# Autodesk Inventor assembly: MIRleft脚四半
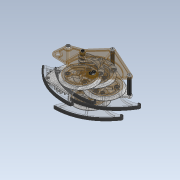
[picture p0: Inventor's stored thumbnail of the model, 180x180]
Saved by Autodesk Inventor 2020.2 (Build 242310000, 310)
## iProperties
Created: 2020-03-11
Part Number: MIRleft脚四半
Document SubType Name: Assembly
Designer: aoyama
Mass: 221.596 g
Surface Area: 1653.51 cm^2
Volume: 107.747 cm^3
Density: 2.05663 g/cm^3
Author: aoyam
## Documents named in this file (38)
- C:\Users\aoyam\Desktop\SRDC_local\Inventor\二年機\Geminiβ\脚\MIR達\MIRleft脚四半.iam
- C:\Users\aoyam\Desktop\SRDC_local\Inventor\二年機\Geminiβ\汎用部品\MIR達\MIRleftワッシャD8d6m0.5.ipt
- C:\Users\aoyam\Desktop\SRDC_local\Inventor\二年機\Geminiβ\汎用部品\MIR達\MIRleftワッシャD7d4m0.5.ipt
- C:\Users\aoyam\Desktop\SRDC_local\Inventor\二年機\Geminiβ\汎用部品\MIR達\MIRleftｍ2歯数17ギアd3.99.ipt
- C:\Users\aoyam\Desktop\SRDC_local\Inventor\二年機\Geminiβ\汎用部品\MIR達\MIRleftスペーサーM3L30アルミ.ipt
- C:\Users\aoyam\Desktop\SRDC_local\Inventor\二年機\Geminiβ\汎用部品\MIR達\MIRleftネジボタンM3L6.ipt
- C:\Users\aoyam\Desktop\SRDC_local\Inventor\二年機\Geminiβ\汎用部品\MIR達\MIRleftネジボタンM3L8.ipt
- C:\Users\aoyam\Desktop\SRDC_local\Inventor\二年機\Geminiβ\汎用部品\MIR達\MIRleftネジボタンM3L10.ipt
- C:\Users\aoyam\Desktop\SRDC_local\Inventor\二年機\Geminiβ\汎用部品\MIR達\MIRleftスペーサーM3L30樹脂.ipt
- C:\Users\aoyam\Desktop\SRDC_local\Inventor\二年機\Geminiβ\汎用部品\MIR達\MIRleftオイレスFd6D8L7.ipt
- C:\Users\aoyam\Desktop\SRDC_local\Inventor\二年機\Geminiβ\汎用部品\MIR達\MIRleftネジアルミM3L6.ipt
- C:\Users\aoyam\Desktop\SRDC_local\Inventor\二年機\Geminiβ\脚\MIR達\MIRleft脚フレーム外側後.ipt
- C:\Users\aoyam\Desktop\SRDC_local\Inventor\二年機\Geminiβ\脚\ネジクランク\MIR達\MIRleft脚一枚.iam
- C:\Users\aoyam\Desktop\SRDC_local\Inventor\二年機\Geminiβ\脚\ネジクランク\MIR達\MIRleftカムL4F.ipt
- C:\Users\aoyam\Desktop\SRDC_local\Inventor\二年機\Geminiβ\汎用部品\MIR達\MIRleftオイレスドライメットFd10D12L3.ipt
- C:\Users\aoyam\Desktop\SRDC_local\Inventor\二年機\Geminiβ\汎用部品\MIR達\MIRleftｍ2歯数25ギアネジ.ipt
- C:\Users\aoyam\Desktop\SRDC_local\Inventor\二年機\Geminiβ\脚\ネジクランク\MIR達\MIRleftカムL3.ipt
- C:\Users\aoyam\Desktop\SRDC_local\Inventor\二年機\Geminiβ\汎用部品\MIR達\MIRleftオイレスドライメットFd10D12L4.ipt
- C:\Users\aoyam\Desktop\SRDC_local\Inventor\二年機\Geminiβ\脚\ネジクランク\MIR達\MIRleftカムL4.ipt
- C:\Users\aoyam\Desktop\SRDC_local\Inventor\二年機\Geminiβ\汎用部品\MIR達\MIRleftネジキャップM3L45.ipt
- C:\Users\aoyam\Desktop\SRDC_local\Inventor\二年機\Geminiβ\汎用部品\MIR達\MIRleftナットナイロンM3.ipt
- C:\Users\aoyam\Desktop\SRDC_local\Inventor\二年機\Geminiβ\汎用部品\MIR達\MIRleftスペーサーM3L40アルミ.ipt
- C:\Users\aoyam\Desktop\SRDC_local\Inventor\二年機\Geminiβ\汎用部品\MIR達\MIRleftネジ超極低頭M3L4.ipt
- C:\Users\aoyam\Desktop\SRDC_local\Inventor\二年機\Geminiβ\汎用部品\MIR達\MIRleftネジキャップM3L15.ipt
- C:\Users\aoyam\Desktop\SRDC_local\Inventor\二年機\Geminiβ\脚\MIR達\MIRleft脚フレーム内側後改.ipt
- C:\Users\aoyam\Desktop\SRDC_local\Inventor\二年機\Geminiβ\汎用部品\ベアリングFd4D11B4.ipt
- C:\Users\aoyam\Desktop\SRDC_local\Inventor\二年機\Geminiβ\汎用部品\オイレスFd6D8L4.ipt
- C:\Users\aoyam\Desktop\SRDC_local\Inventor\二年機\Geminiβ\汎用部品\ベアリングFd6D12B4.ipt
- C:\Users\aoyam\Desktop\SRDC_local\Inventor\二年機\Geminiβ\汎用部品\ワッシャD8d6m0.5.ipt
- C:\Users\aoyam\Desktop\SRDC_local\Inventor\二年機\Geminiβ\汎用部品\ｍ2歯数14ギアd12.ipt
- C:\Users\aoyam\Desktop\SRDC_local\Inventor\二年機\Geminiβ\汎用部品\ワッシャD10d6m0.3.ipt
- C:\Users\aoyam\Desktop\SRDC_local\Inventor\二年機\Geminiβ\汎用部品\オイレス外径8内径6L3.ipt
- C:\Users\aoyam\Desktop\SRDC_local\Inventor\二年機\Geminiβ\脚\MIRright脚ギアトレイン2.ipt
- C:\Users\aoyam\Desktop\SRDC_local\Inventor\二年機\Geminiβ\汎用部品\スペーサー中空M3L5樹脂.ipt
- C:\Users\aoyam\Desktop\SRDC_local\Inventor\二年機\Geminiβ\汎用部品\スペーサー中空M3L4樹脂.ipt
- C:\Users\aoyam\Desktop\SRDC_local\Inventor\二年機\Geminiβ\汎用部品\ネジ皿M3L8.ipt
- C:\Users\aoyam\Desktop\SRDC_local\Inventor\二年機\Geminiβ\汎用部品\ポリスラd6D14t0.25.ipt
- C:\Users\aoyam\Desktop\SRDC_local\Inventor\二年機\Geminiβ\汎用部品\平行ピンD4L12.ipt
## Components (61 placed, 37 different names)
1. MIRleftワッシャD7d4m0.5:1 — 挿入:9, 挿入:82
2. MIRleftｍ2歯数17ギアd3.99:1 — 挿入:9, 挿入:11
3. MIRleftワッシャD7d4m0.5:2 — 挿入:11, 挿入:81
4. MIRleftスペーサーM3L30アルミ:1 — 挿入:93, メイト:9, メイト:10, メイト:11, メイト:12, メイト:9, 挿入:73
5. MIRleftネジボタンM3L6:1 — 挿入:74
6. MIRleftネジボタンM3L8:1 — 挿入:97, メイト:9
7. MIRleftネジボタンM3L10:1 — 挿入:99
8. MIRleftネジボタンM3L10:2 — 挿入:97
9. MIRleftネジボタンM3L10:3 — 挿入:98
10. MIRleftスペーサーM3L30樹脂:1 — 挿入:71
11. MIRleftスペーサーM3L30樹脂:2 — 挿入:72, 挿入:77
12. MIRleftオイレスFd6D8L7:1 — 挿入:136, 挿入:137
13. MIRleftオイレスFd6D8L7:2 — 挿入:134
14. MIRleftオイレスFd6D8L7:3 — 挿入:135
15. MIRleftオイレスFd6D8L7:4 — 挿入:133
16. MIRleftワッシャD8d6m0.5:3 — 挿入:93, 挿入:129
17. MIRleftワッシャD8d6m0.5:4 — 挿入:130
18. MIRleftワッシャD8d6m0.5:5 — 挿入:129
19. MIRleftネジアルミM3L6:1 — 挿入:75
20. MIRleftネジアルミM3L6:2 — 挿入:76
21. MIRleftネジアルミM3L6:3 — 挿入:98
22. MIRleftネジアルミM3L6:4 — 挿入:99
23. MIRleft脚フレーム外側後:1 — 挿入:99, 挿入:98, 挿入:97, メイト:1, 挿入:111, 挿入:124, 挿入:77
24. MIRleft脚一枚:1 [sub-assembly] — 挿入:136, メイト:9, メイト:1, 挿入:104, 挿入:103, 挿入:110, 挿入:109
25. MIRleft脚一枚:2 [sub-assembly] — 挿入:135, メイト:10, 挿入:104, 挿入:103, 挿入:106, 挿入:105
26. MIRleft脚一枚:3 [sub-assembly] — 挿入:134, メイト:11, 挿入:106, 挿入:105, 挿入:108, 挿入:107
27. MIRleft脚一枚:4 [sub-assembly] — 挿入:133, メイト:12, 挿入:108, 挿入:107, メイト:6, メイト:7
28. MIRleftカムL4F:1 — 挿入:111, 挿入:110, 挿入:109, 挿入:112, 挿入:119, 挿入:120
29. MIRleftオイレスドライメットFd10D12L3:1 — 挿入:112
30. MIRleftｍ2歯数25ギアネジ:1 — メイト:6, 挿入:114, 挿入:116, 挿入:115, 挿入:78
31. MIRleftオイレスドライメットFd10D12L3:2 — 挿入:114
32. MIRleftカムL3:1 — 挿入:116, 挿入:115, 挿入:121, 挿入:122
33. MIRleftオイレスドライメットFd10D12L4:1 — 挿入:118, 挿入:78, 挿入:79
34. MIRleftカムL4:1 — メイト:7, 挿入:118
35. MIRleftネジキャップM3L45:1 — 挿入:119, メイト:10
36. MIRleftネジキャップM3L45:2 — 挿入:120
37. MIRleftナットナイロンM3:1 — 挿入:121, メイト:8, メイト:10
38. MIRleftナットナイロンM3:2 — メイト:8, 挿入:122
39. MIRleftスペーサーM3L40アルミ:1 — 挿入:124, 挿入:127, 挿入:100
40. MIRleftネジ超極低頭M3L4:1 — 挿入:127
41. MIRleftワッシャD8d6m0.5:6 — 挿入:137, 挿入:130
42. MIRleftネジキャップM3L15:1 — 挿入:101
43. MIRleft脚フレーム内側後改:1 — 挿入:71, 挿入:72, 挿入:73, 挿入:74, 挿入:75, 挿入:76, 挿入:79, 挿入:80, 挿入:83, 挿入:90, 挿入:91, 挿入:92, 挿入:93, 挿入:102
44. ベアリングFd4D11B4:1 — 挿入:82, 挿入:105
45. ベアリングFd4D11B4:2 — 挿入:80, 挿入:81
46. オイレスFd6D8L4:1 — 挿入:83, 挿入:84
47. ベアリングFd6D12B4:1 — 挿入:85, 挿入:86, 挿入:87
48. ワッシャD8d6m0.5:1 — 挿入:84, 挿入:85
49. ｍ2歯数14ギアd12:1 — 挿入:86
50. ワッシャD10d6m0.3:1 — 挿入:87, 挿入:88
51. オイレス外径8内径6L3:1 — 挿入:88, 挿入:89, 挿入:104
52. MIRright脚ギアトレイン2:1 — 挿入:89, 挿入:94, 挿入:95, 挿入:96, 挿入:97, 挿入:98, 挿入:99, 挿入:101
53. スペーサー中空M3L5樹脂:1 — 挿入:90, 挿入:94
54. スペーサー中空M3L5樹脂:2 — 挿入:91, 挿入:96
55. スペーサー中空M3L5樹脂:3 — 挿入:92, 挿入:95
56. スペーサー中空M3L5樹脂:4 — 挿入:93
57. スペーサー中空M3L4樹脂:1 — 挿入:100
58. ネジ皿M3L8:1 — 挿入:102
59. ポリスラd6D14t0.25:1 — 挿入:103
60. ポリスラd6D14t0.25:2 — 挿入:103, 挿入:104
61. 平行ピンD4L12:1 — 挿入:105
## Relationships (78: Insert 68, Mate 10)
- 挿入:9 [Insert]: MIRleftワッシャD7d4m0.5:1 ↔ MIRleftｍ2歯数17ギアd3.99:1
- 挿入:11 [Insert]: MIRleftｍ2歯数17ギアd3.99:1 ↔ MIRleftワッシャD7d4m0.5:2
- 挿入:93 [Insert]: MIRleftスペーサーM3L30アルミ:1 ↔ MIRleftワッシャD8d6m0.5:3
- 挿入:129 [Insert]: MIRleftワッシャD8d6m0.5:3 ↔ MIRleftワッシャD8d6m0.5:5
- 挿入:99 [Insert]: MIRleftネジアルミM3L6:4 ↔ MIRleft脚フレーム外側後:1
- 挿入:98 [Insert]: MIRleftネジアルミM3L6:3 ↔ MIRleft脚フレーム外側後:1
- 挿入:97 [Insert]: MIRleftネジボタンM3L8:1 ↔ MIRleft脚フレーム外側後:1
- 挿入:136 [Insert]: MIRleftオイレスFd6D8L7:1 ↔ MIRleft脚一枚:1
- メイト:9 [Mate]: MIRleftスペーサーM3L30アルミ:1 ↔ MIRleft脚一枚:1
- メイト:1 [Mate] (1 mm): MIRleft脚フレーム外側後:1 ↔ MIRleft脚一枚:1
- 挿入:135 [Insert]: MIRleftオイレスFd6D8L7:3 ↔ MIRleft脚一枚:2
- メイト:10 [Mate]: MIRleftスペーサーM3L30アルミ:1 ↔ MIRleft脚一枚:2
- 挿入:104 [Insert]: MIRleft脚一枚:1 ↔ MIRleft脚一枚:2
- 挿入:103 [Insert]: MIRleft脚一枚:1 ↔ MIRleft脚一枚:2
- 挿入:134 [Insert]: MIRleftオイレスFd6D8L7:2 ↔ MIRleft脚一枚:3
- メイト:11 [Mate]: MIRleftスペーサーM3L30アルミ:1 ↔ MIRleft脚一枚:3
- 挿入:106 [Insert]: MIRleft脚一枚:2 ↔ MIRleft脚一枚:3
- 挿入:105 [Insert]: MIRleft脚一枚:2 ↔ MIRleft脚一枚:3
- 挿入:133 [Insert]: MIRleftオイレスFd6D8L7:4 ↔ MIRleft脚一枚:4
- メイト:12 [Mate]: MIRleftスペーサーM3L30アルミ:1 ↔ MIRleft脚一枚:4
- 挿入:108 [Insert]: MIRleft脚一枚:3 ↔ MIRleft脚一枚:4
- 挿入:107 [Insert]: MIRleft脚一枚:3 ↔ MIRleft脚一枚:4
- 挿入:111 [Insert]: MIRleft脚フレーム外側後:1 ↔ MIRleftカムL4F:1
- 挿入:110 [Insert]: MIRleft脚一枚:1 ↔ MIRleftカムL4F:1
- 挿入:109 [Insert]: MIRleft脚一枚:1 ↔ MIRleftカムL4F:1
- 挿入:112 [Insert]: MIRleftカムL4F:1 ↔ MIRleftオイレスドライメットFd10D12L3:1
- メイト:6 [Mate]: MIRleft脚一枚:4 ↔ MIRleftｍ2歯数25ギアネジ:1
- 挿入:114 [Insert]: MIRleftｍ2歯数25ギアネジ:1 ↔ MIRleftオイレスドライメットFd10D12L3:2
- 挿入:116 [Insert]: MIRleftｍ2歯数25ギアネジ:1 ↔ MIRleftカムL3:1
- 挿入:115 [Insert]: MIRleftｍ2歯数25ギアネジ:1 ↔ MIRleftカムL3:1
- メイト:7 [Mate]: MIRleft脚一枚:4 ↔ MIRleftカムL4:1
- 挿入:118 [Insert]: MIRleftオイレスドライメットFd10D12L4:1 ↔ MIRleftカムL4:1
- 挿入:119 [Insert]: MIRleftカムL4F:1 ↔ MIRleftネジキャップM3L45:1
- 挿入:120 [Insert]: MIRleftカムL4F:1 ↔ MIRleftネジキャップM3L45:2
- 挿入:121 [Insert]: MIRleftカムL3:1 ↔ MIRleftナットナイロンM3:1
- メイト:8 [Mate]: MIRleftナットナイロンM3:1 ↔ MIRleftナットナイロンM3:2
- 挿入:122 [Insert]: MIRleftカムL3:1 ↔ MIRleftナットナイロンM3:2
- 挿入:124 [Insert] (3 mm): MIRleft脚フレーム外側後:1 ↔ MIRleftスペーサーM3L40アルミ:1
- 挿入:127 [Insert]: MIRleftスペーサーM3L40アルミ:1 ↔ MIRleftネジ超極低頭M3L4:1
- 挿入:137 [Insert]: MIRleftオイレスFd6D8L7:1 ↔ MIRleftワッシャD8d6m0.5:6
- 挿入:130 [Insert]: MIRleftワッシャD8d6m0.5:4 ↔ MIRleftワッシャD8d6m0.5:6
- メイト:9 [Mate]: MIRleftスペーサーM3L30アルミ:1 ↔ MIRleftネジボタンM3L8:1
- 挿入:71 [Insert]: MIRleftスペーサーM3L30樹脂:1 ↔ MIRleft脚フレーム内側後改:1
- 挿入:72 [Insert]: MIRleftスペーサーM3L30樹脂:2 ↔ MIRleft脚フレーム内側後改:1
- 挿入:73 [Insert]: MIRleftスペーサーM3L30アルミ:1 ↔ MIRleft脚フレーム内側後改:1
- 挿入:74 [Insert]: MIRleftネジボタンM3L6:1 ↔ MIRleft脚フレーム内側後改:1
- 挿入:75 [Insert]: MIRleftネジアルミM3L6:1 ↔ MIRleft脚フレーム内側後改:1
- 挿入:76 [Insert]: MIRleftネジアルミM3L6:2 ↔ MIRleft脚フレーム内側後改:1
- メイト:10 [Mate]: MIRleftネジキャップM3L45:1 ↔ MIRleftナットナイロンM3:1
- 挿入:77 [Insert]: MIRleftスペーサーM3L30樹脂:2 ↔ MIRleft脚フレーム外側後:1
- 挿入:78 [Insert]: MIRleftｍ2歯数25ギアネジ:1 ↔ MIRleftオイレスドライメットFd10D12L4:1
- 挿入:79 [Insert]: MIRleftオイレスドライメットFd10D12L4:1 ↔ MIRleft脚フレーム内側後改:1
- 挿入:80 [Insert]: MIRleft脚フレーム内側後改:1 ↔ ベアリングFd4D11B4:2
- 挿入:81 [Insert]: MIRleftワッシャD7d4m0.5:2 ↔ ベアリングFd4D11B4:2
- 挿入:82 [Insert]: MIRleftワッシャD7d4m0.5:1 ↔ ベアリングFd4D11B4:1
- 挿入:83 [Insert]: MIRleft脚フレーム内側後改:1 ↔ オイレスFd6D8L4:1
- 挿入:84 [Insert]: オイレスFd6D8L4:1 ↔ ワッシャD8d6m0.5:1
- 挿入:85 [Insert]: ベアリングFd6D12B4:1 ↔ ワッシャD8d6m0.5:1
- 挿入:86 [Insert]: ベアリングFd6D12B4:1 ↔ ｍ2歯数14ギアd12:1
- 挿入:87 [Insert]: ベアリングFd6D12B4:1 ↔ ワッシャD10d6m0.3:1
- 挿入:88 [Insert]: ワッシャD10d6m0.3:1 ↔ オイレス外径8内径6L3:1
- 挿入:89 [Insert]: オイレス外径8内径6L3:1 ↔ MIRright脚ギアトレイン2:1
- 挿入:90 [Insert]: MIRleft脚フレーム内側後改:1 ↔ スペーサー中空M3L5樹脂:1
- 挿入:91 [Insert]: MIRleft脚フレーム内側後改:1 ↔ スペーサー中空M3L5樹脂:2
- 挿入:92 [Insert]: MIRleft脚フレーム内側後改:1 ↔ スペーサー中空M3L5樹脂:3
- 挿入:93 [Insert]: MIRleft脚フレーム内側後改:1 ↔ スペーサー中空M3L5樹脂:4
- 挿入:94 [Insert]: MIRright脚ギアトレイン2:1 ↔ スペーサー中空M3L5樹脂:1
- 挿入:95 [Insert]: MIRright脚ギアトレイン2:1 ↔ スペーサー中空M3L5樹脂:3
- 挿入:96 [Insert]: MIRright脚ギアトレイン2:1 ↔ スペーサー中空M3L5樹脂:2
- 挿入:97 [Insert]: MIRleftネジボタンM3L10:2 ↔ MIRright脚ギアトレイン2:1
- 挿入:98 [Insert]: MIRleftネジボタンM3L10:3 ↔ MIRright脚ギアトレイン2:1
- 挿入:99 [Insert]: MIRleftネジボタンM3L10:1 ↔ MIRright脚ギアトレイン2:1
- 挿入:100 [Insert]: MIRleftスペーサーM3L40アルミ:1 ↔ スペーサー中空M3L4樹脂:1
- 挿入:101 [Insert]: MIRleftネジキャップM3L15:1 ↔ MIRright脚ギアトレイン2:1
- 挿入:102 [Insert]: MIRleft脚フレーム内側後改:1 ↔ ネジ皿M3L8:1
- 挿入:103 [Insert]: ポリスラd6D14t0.25:1 ↔ ポリスラd6D14t0.25:2
- 挿入:104 [Insert]: オイレス外径8内径6L3:1 ↔ ポリスラd6D14t0.25:2
- 挿入:105 [Insert]: ベアリングFd4D11B4:1 ↔ 平行ピンD4L12:1
